# Autodesk Inventor assembly: table
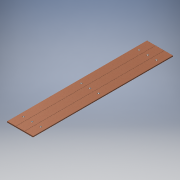
[picture p0: Inventor's stored thumbnail of the model, 180x180]
Saved by Autodesk Inventor 2019 (Build 230136000, 136)
## iProperties
Created: 2019-02-27
Part Number: table
Document SubType Name: Assembly
Designer: gaincarlo
Author: gaincarlo
## Documents named in this file (4)
- D:\Giancarlo Bacchio\Documenti\00 - Progetti\30-Inventor\LaPanca-Baraca\table.iam
- D:\Giancarlo Bacchio\Documenti\00 - Progetti\30-Inventor\LaPanca-Baraca\doga_long1.ipt
- D:\Giancarlo Bacchio\Documenti\00 - Progetti\30-Inventor\LaPanca-Baraca\support3.ipt
- D:\Giancarlo Bacchio\Documenti\Inventor\Content Center Files\R2019\en-US\GB_T 15-88\Bolt GB_T 15 M8 x 35.ipt
## Components (15 placed, 3 different names)
1. doga_long1:1 — Mate:1, Mate:4, Mate:5
2. doga_long1:2 — Mate:2
3. doga_long1:3 — Mate:3
4. support3:1 — Mate:1, Mate:2, Mate:3
5. support3:2
6. support3:3
7. Bolt GB/T 15-1988 M8x35:1 — Mate:4, Mate:5
8. Bolt GB/T 15-1988 M8x35:2
9. Bolt GB/T 15-1988 M8x35:3
10. Bolt GB/T 15-1988 M8x35:4
11. Bolt GB/T 15-1988 M8x35:5
12. Bolt GB/T 15-1988 M8x35:6
13. Bolt GB/T 15-1988 M8x35:7
14. Bolt GB/T 15-1988 M8x35:8
15. Bolt GB/T 15-1988 M8x35:9
## Component patterns: (3 elements, first: doga_long1:1), (3 elements, first: support3:1), (3 elements, first: Bolt GB/T 15-1988 M8x35:1), Component Pattern 2:2 (3 elements), Component Pattern 2:3 (3 elements)
## Relationships (5: Mate 5)
- Mate:1: doga_long1:1 ↔ support3:1
- Mate:2: doga_long1:2 ↔ support3:1
- Mate:3: doga_long1:3 ↔ support3:1
- Mate:4: doga_long1:1 ↔ Bolt GB/T 15-1988 M8x35:1
- Mate:5: doga_long1:1 ↔ Bolt GB/T 15-1988 M8x35:1
